# Autodesk Inventor assembly: spinner
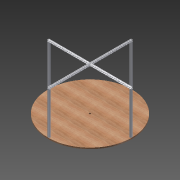
[picture p0: Inventor's stored thumbnail of the model, 180x180]
Saved by Autodesk Inventor 2013 (Build 170138000, 138)
## iProperties
Created: 2013-04-07
Part Number: spinner
Document SubType Name: Assembly
Designer: Chris
Mass: 23731.6 g
Surface Area: 35376.3 cm^2
Volume: 23731.6 cm^3
Density: 1 g/cm^3
Author: Chris
## Documents named in this file (6)
- C:\Users\Chris\Documents\Inventor\Redbull-2013\8020\spinner.iam
- C:\Users\Chris\Documents\Inventor\Redbull-2013\crazyness\bottom.ipt
- C:\Users\Chris\Documents\Inventor\Redbull-2013\8020\8020-1010-24-in.ipt
- C:\Users\Chris\Documents\Inventor\Redbull-2013\8020\8020-1010-48-in.ipt
- C:\Users\Chris\Documents\Inventor\Redbull-2013\8020\8020-1010-23-5-in.ipt
- C:\Users\Chris\Documents\Inventor\Redbull-2013\Imported Components\RushGears_ap214_S2056\RushGears_ap214_S2056.ipt
## Components (9 placed, 5 different names)
1. bottom:1 — Insert:1, Insert:2, Insert:3, Insert:4, Insert:5
2. 8020-1010-24-in:1 — Insert:1, Flush:1
3. 8020-1010-24-in:2 — Insert:2, Flush:1, Mate:1, Flush:3, Flush:4
4. 8020-1010-24-in:3 — Insert:4, Flush:2, Flush:7, Mate:3, Flush:8
5. 8020-1010-24-in:4 — Insert:3, Flush:2, Flush:5, Flush:6, Mate:2
6. 8020-1010-48-in:1 — Mate:1, Flush:3, Flush:4
7. 8020-1010-23-5-in:1 — Flush:5, Flush:6, Mate:2
8. 8020-1010-23-5-in:2 — Flush:7, Mate:3, Flush:8
9. RushGears_ap214_S2056:1 — Insert:5
## Relationships (16: Flush 8, Insert 5, Mate 3)
- Insert:1: bottom:1 ↔ 8020-1010-24-in:1
- Insert:2: bottom:1 ↔ 8020-1010-24-in:2
- Flush:1: 8020-1010-24-in:1 ↔ 8020-1010-24-in:2
- Insert:3: bottom:1 ↔ 8020-1010-24-in:4
- Insert:4: bottom:1 ↔ 8020-1010-24-in:3
- Flush:2: 8020-1010-24-in:3 ↔ 8020-1010-24-in:4
- Mate:1: 8020-1010-24-in:2 ↔ 8020-1010-48-in:1
- Flush:3: 8020-1010-24-in:2 ↔ 8020-1010-48-in:1
- Flush:4: 8020-1010-24-in:2 ↔ 8020-1010-48-in:1
- Flush:5: 8020-1010-24-in:4 ↔ 8020-1010-23-5-in:1
- Flush:6: 8020-1010-24-in:4 ↔ 8020-1010-23-5-in:1
- Mate:2: 8020-1010-24-in:4 ↔ 8020-1010-23-5-in:1
- Flush:7: 8020-1010-24-in:3 ↔ 8020-1010-23-5-in:2
- Mate:3: 8020-1010-24-in:3 ↔ 8020-1010-23-5-in:2
- Flush:8: 8020-1010-24-in:3 ↔ 8020-1010-23-5-in:2
- Insert:5: bottom:1 ↔ RushGears_ap214_S2056:1
